# Autodesk Inventor assembly: bellows_latest
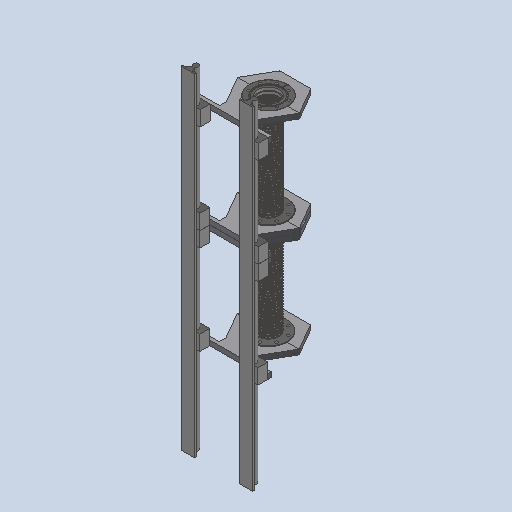
[picture p0: Inventor's stored thumbnail of the model, 512x512]
Saved by Autodesk Inventor 2026.3 (Build 303398000, 398)
## iProperties
Created: 2026-06-04
Part Number: bellows_latest
Document SubType Name: Assembly
Designer: shusu
Author: shusu
## Documents named in this file (3)
- C:\Users\shusu\OneDrive - Kyoto University\デスクトップ\蓮尾研\ベローズ設計\bellows_latest.iam
- C:\Users\shusu\OneDrive - Kyoto University\デスクトップ\蓮尾研\ベローズ設計\bellows_kihon.iam
- C:\Users\shusu\OneDrive - Kyoto University\デスクトップ\蓮尾研\ベローズ設計\rail.ipt
## Components (4 placed, 2 different names)
1. bellows_kihon:1 [sub-assembly] — メイト:1, 角度:1, 角度:2, 挿入:1, 挿入:2
2. bellows_kihon:2 [sub-assembly] — メイト:1
3. rail:1 — 角度:1, 挿入:1
4. rail:2 — 角度:2, 挿入:2
## Relationships (5: Angle 2, Insert 2, Mate 1)
- メイト:1 [Mate]: bellows_kihon:1 ↔ bellows_kihon:2
- 角度:1 [Angle] (0 deg): bellows_kihon:1 ↔ rail:1
- 角度:2 [Angle] (0 deg): bellows_kihon:1 ↔ rail:2
- 挿入:1 [Insert] (-100 mm): bellows_kihon:1 ↔ rail:1
- 挿入:2 [Insert] (-100 mm): bellows_kihon:1 ↔ rail:2
